# Autodesk Inventor assembly: sekkeiseisakuron
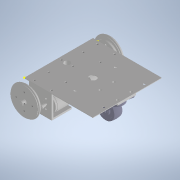
[picture p0: Inventor's stored thumbnail of the model, 180x180]
Saved by Autodesk Inventor 2022.1 (Build 261234020, 234B)
## iProperties
Created: 2021-10-16
Part Number: sekkeiseisakuron
Document SubType Name: Assembly
Designer: gilte
Author: gilte
## Documents named in this file (18)
- C:\Users\gilte\Documents\Inventor\kadai3\sekkeiseisakuron.iam
- C:\Users\gilte\Documents\Inventor\kadai3\RD002_フレーム.ipt
- C:\Users\gilte\Documents\Inventor\kadai3\RD004_スペーサ.ipt
- C:\Users\gilte\Documents\Inventor\kadai3\RD003_キャスタ420G-R32.ipt
- C:\Users\gilte\Documents\Inventor\kadai3\RD006_ギヤボックス左.ipt
- C:\Users\gilte\Documents\Inventor\kadai3\RD007_ギヤボックス右.ipt
- C:\Users\gilte\Documents\Inventor\kadai3\RD005_ペンホルダ.ipt
- C:\Users\gilte\Documents\Inventor\kadai3\RD014_ストッパ.ipt
- C:\Users\gilte\Documents\Inventor\kadai3\RD015_シャフト.ipt
- C:\Users\gilte\Documents\Inventor\kadai3\RD008_モータ(DMN29).ipt
- C:\Users\gilte\Documents\Inventor\kadai3\RD009_ギアDS0.5-12.ipt
- C:\Users\gilte\Documents\Inventor\kadai3\RD020_ワッシャ.ipt
- C:\Users\gilte\Documents\Inventor\kadai3\RD019_ブッシュ80F-0305改.ipt
- C:\Users\gilte\Documents\Inventor\kadai3\RD010_ギアDS0.5-80.ipt
- C:\Users\gilte\Documents\Inventor\kadai3\RD011_ギア用ブッシュ.ipt
- C:\Users\gilte\Documents\Inventor\kadai3\RD018_ブッシュ80F-0305.ipt
- C:\Users\gilte\Documents\Inventor\kadai3\RD012_ホイール.ipt
- C:\Users\gilte\Documents\Inventor\kadai3\RD013_オーリング.ipt
## Components (30 placed, 17 different names)
1. RD002_フレーム:1 — 挿入:1, 挿入:2, 挿入:9, 挿入:10, 挿入:28, 挿入:29, 挿入:30
2. RD004_スペーサ:1 — 挿入:1, 挿入:2, 挿入:3, 挿入:4
3. RD003_キャスタ420G-R32:1 — 挿入:3, 挿入:4
4. RD005_ペンホルダ:1 — 挿入:9, 挿入:10
5. RD014_ストッパ:2 — 挿入:47
6. RD014_ストッパ:4 — 挿入:48
7. RD010_ギアDS0.5-80:1 — 挿入:25
8. RD011_ギア用ブッシュ:1 — 挿入:25, 挿入:42, 挿入:45
9. RD006_ギヤボックス左:1 — 挿入:28, 挿入:29, 挿入:32, 挿入:33, 挿入:36, 挿入:51, 挿入:52
10. RD007_ギヤボックス右:1 — 挿入:30, 挿入:31, 挿入:37, 挿入:49, 挿入:50
11. RD014_ストッパ:5 — 挿入:31, 挿入:35
12. RD014_ストッパ:6 — 挿入:32, 挿入:33, 挿入:34
13. RD015_シャフト:1 — 挿入:34
14. RD015_シャフト:2 — 挿入:35
15. RD020_ワッシャ:1 — 挿入:36, 挿入:39
16. RD020_ワッシャ:2 — 挿入:37, 挿入:38
17. RD019_ブッシュ80F-0305改:1 — 挿入:38, 挿入:42
18. RD019_ブッシュ80F-0305改:2 — 挿入:39, 挿入:41
19. RD010_ギアDS0.5-80:2 — 挿入:40
20. RD011_ギア用ブッシュ:2 — 挿入:40, 挿入:41, 挿入:46
21. RD018_ブッシュ80F-0305:1 — 挿入:44, 挿入:46, 挿入:47
22. RD018_ブッシュ80F-0305:2 — 挿入:43, 挿入:45, 挿入:48
23. RD012_ホイール:1 — 挿入:43, メイト:1, 正接:1
24. RD012_ホイール:2 — 挿入:44, メイト:2, 正接:2
25. RD008_モータ(DMN29):1 — 挿入:51, 挿入:52, 挿入:53
26. RD008_モータ(DMN29):2 — 挿入:49, 挿入:50, 挿入:54
27. RD009_ギアDS0.5-12:1 — 挿入:54
28. RD009_ギアDS0.5-12:2 — 挿入:53
29. RD013_オーリング:1 — メイト:1, 正接:1
30. RD013_オーリング:2 — メイト:2, 正接:2
## Relationships (38: Insert 34, Mate 2, Tangent 2)
- 挿入:1 [Insert]: RD002_フレーム:1 ↔ RD004_スペーサ:1
- 挿入:2 [Insert]: RD002_フレーム:1 ↔ RD004_スペーサ:1
- 挿入:3 [Insert]: RD004_スペーサ:1 ↔ RD003_キャスタ420G-R32:1
- 挿入:4 [Insert]: RD004_スペーサ:1 ↔ RD003_キャスタ420G-R32:1
- 挿入:9 [Insert]: RD002_フレーム:1 ↔ RD005_ペンホルダ:1
- 挿入:10 [Insert]: RD002_フレーム:1 ↔ RD005_ペンホルダ:1
- 挿入:25 [Insert]: RD010_ギアDS0.5-80:1 ↔ RD011_ギア用ブッシュ:1
- 挿入:28 [Insert]: RD002_フレーム:1 ↔ RD006_ギヤボックス左:1
- 挿入:29 [Insert]: RD002_フレーム:1 ↔ RD006_ギヤボックス左:1
- 挿入:30 [Insert]: RD002_フレーム:1 ↔ RD007_ギヤボックス右:1
- 挿入:31 [Insert]: RD007_ギヤボックス右:1 ↔ RD014_ストッパ:5
- 挿入:32 [Insert]: RD006_ギヤボックス左:1 ↔ RD014_ストッパ:6
- 挿入:33 [Insert]: RD006_ギヤボックス左:1 ↔ RD014_ストッパ:6
- 挿入:34 [Insert]: RD014_ストッパ:6 ↔ RD015_シャフト:1
- 挿入:35 [Insert]: RD014_ストッパ:5 ↔ RD015_シャフト:2
- 挿入:36 [Insert]: RD006_ギヤボックス左:1 ↔ RD020_ワッシャ:1
- 挿入:37 [Insert]: RD007_ギヤボックス右:1 ↔ RD020_ワッシャ:2
- 挿入:38 [Insert]: RD020_ワッシャ:2 ↔ RD019_ブッシュ80F-0305改:1
- 挿入:39 [Insert]: RD020_ワッシャ:1 ↔ RD019_ブッシュ80F-0305改:2
- 挿入:40 [Insert]: RD010_ギアDS0.5-80:2 ↔ RD011_ギア用ブッシュ:2
- 挿入:41 [Insert]: RD019_ブッシュ80F-0305改:2 ↔ RD011_ギア用ブッシュ:2
- 挿入:42 [Insert]: RD011_ギア用ブッシュ:1 ↔ RD019_ブッシュ80F-0305改:1
- 挿入:43 [Insert]: RD018_ブッシュ80F-0305:2 ↔ RD012_ホイール:1
- 挿入:44 [Insert]: RD018_ブッシュ80F-0305:1 ↔ RD012_ホイール:2
- 挿入:45 [Insert]: RD011_ギア用ブッシュ:1 ↔ RD018_ブッシュ80F-0305:2
- 挿入:46 [Insert]: RD011_ギア用ブッシュ:2 ↔ RD018_ブッシュ80F-0305:1
- 挿入:47 [Insert]: RD014_ストッパ:2 ↔ RD018_ブッシュ80F-0305:1
- 挿入:48 [Insert]: RD014_ストッパ:4 ↔ RD018_ブッシュ80F-0305:2
- 挿入:49 [Insert]: RD007_ギヤボックス右:1 ↔ RD008_モータ(DMN29):2
- 挿入:50 [Insert]: RD007_ギヤボックス右:1 ↔ RD008_モータ(DMN29):2
- 挿入:51 [Insert]: RD006_ギヤボックス左:1 ↔ RD008_モータ(DMN29):1
- 挿入:52 [Insert]: RD006_ギヤボックス左:1 ↔ RD008_モータ(DMN29):1
- 挿入:53 [Insert]: RD008_モータ(DMN29):1 ↔ RD009_ギアDS0.5-12:2
- 挿入:54 [Insert]: RD008_モータ(DMN29):2 ↔ RD009_ギアDS0.5-12:1
- メイト:1 [Mate]: RD012_ホイール:1 ↔ RD013_オーリング:1
- 正接:1 [Tangent]: RD012_ホイール:1 ↔ RD013_オーリング:1
- メイト:2 [Mate]: RD012_ホイール:2 ↔ RD013_オーリング:2
- 正接:2 [Tangent]: RD012_ホイール:2 ↔ RD013_オーリング:2
